# Autodesk Inventor assembly: T-Frame
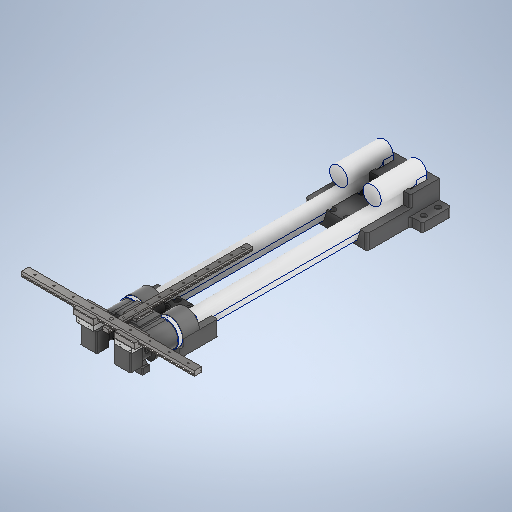
[picture p0: Inventor's stored thumbnail of the model, 512x512]
Saved by Autodesk Inventor 2026.2 (Build 302298010, 298A)
## iProperties
Created: 2026-03-27
Part Number: T-Frame
Document SubType Name: Assembly
Designer: chanh
Author: chanh
## Documents named in this file (15)
- C:\Users\chanh\내 드라이브\교과공부\2026년 1학기 (4학년 1학기)\01창의제품설계\CLOSE_hardware\02하체\도면\T-Frame.iam
- C:\Users\chanh\내 드라이브\교과공부\2026년 1학기 (4학년 1학기)\01창의제품설계\CLOSE_hardware\02하체\Linear Motor Bar (T-Frame).ipt
- C:\Users\chanh\내 드라이브\교과공부\2026년 1학기 (4학년 1학기)\01창의제품설계\CLOSE_hardware\02하체\Linear Motor (T-Frame).ipt
- C:\Users\chanh\내 드라이브\교과공부\2026년 1학기 (4학년 1학기)\01창의제품설계\CLOSE_hardware\02하체\Linear Motor Rear Braket.ipt
- C:\Users\chanh\내 드라이브\교과공부\2026년 1학기 (4학년 1학기)\01창의제품설계\CLOSE_hardware\02하체\Linear Motor Front Braket.ipt
- C:\Users\chanh\내 드라이브\교과공부\2026년 1학기 (4학년 1학기)\01창의제품설계\CLOSE_hardware\02하체\LMF20UU.ipt
- C:\Users\chanh\내 드라이브\교과공부\2026년 1학기 (4학년 1학기)\01창의제품설계\CLOSE_hardware\02하체\MGN15C Cart.ipt
- C:\Users\chanh\내 드라이브\교과공부\2026년 1학기 (4학년 1학기)\01창의제품설계\CLOSE_hardware\02하체\MGN15 Rail.ipt
- C:\Users\chanh\내 드라이브\교과공부\2026년 1학기 (4학년 1학기)\01창의제품설계\CLOSE_hardware\02하체\Linear Motor Mount Right.ipt
- C:\Users\chanh\내 드라이브\교과공부\2026년 1학기 (4학년 1학기)\01창의제품설계\CLOSE_hardware\02하체\Linear Motor Mount Left.ipt
- C:\Users\chanh\내 드라이브\교과공부\2026년 1학기 (4학년 1학기)\01창의제품설계\CLOSE_hardware\02하체\LM Cart Braket.ipt
- C:\Users\chanh\내 드라이브\교과공부\2026년 1학기 (4학년 1학기)\01창의제품설계\CLOSE_hardware\02하체\Space Craft Braket.ipt
- C:\Users\chanh\내 드라이브\교과공부\2026년 1학기 (4학년 1학기)\01창의제품설계\CLOSE_hardware\02하체\LM20UU.ipt
- C:\Users\chanh\내 드라이브\교과공부\2026년 1학기 (4학년 1학기)\01창의제품설계\CLOSE_hardware\02하체\MGN12C Cart.ipt
- C:\Users\chanh\내 드라이브\교과공부\2026년 1학기 (4학년 1학기)\01창의제품설계\CLOSE_hardware\02하체\MGN12 Rail.ipt
## Components (20 placed, 14 different names)
1. MGN15C Cart:1 — Slider:2, Rigid:8
2. MGN15 Rail:1 — Slider:1, Slider:2, Rotational:1
3. MGN15C Cart:2 — Slider:1, Flush:67, Flush:68, Mate:67
4. Linear Motor Mount Right:1 — Rigid:7, Mate:72
5. Linear Motor Mount Left:1 — Rigid:9, Mate:73
6. LM Cart Braket:1 — Flush:67, Flush:68, Mate:67, Mate:72
7. LM Cart Braket:2 — Rigid:8, Mate:73
8. Space Craft Braket:1 — Rigid:10, Rigid:11, Rigid:13
9. LM20UU:1 — Rigid:10, Mate:69
10. LM20UU:2 — Rigid:11, Mate:68
11. MGN12C Cart:1 — Rigid:13, Slider:3
12. MGN12 Rail:1 — Slider:3, Rotational:1
13. Linear Motor Front Braket:1 — Flush:56, Rigid:5, Rigid:6
14. LMF20UU:1 — Rigid:5
15. LMF20UU:2 — Rigid:6
16. Linear Motor (T-Frame):1 — Mate:32, Angle:2, T자 왼쪽 거리, Flush:53
17. Linear Motor Bar (T-Frame):1 — Mate:32, Angle:2, T자 왼쪽 거리, Rigid:7, Mate:69
18. Linear Motor (T-Frame):2 — T자 오른쪽 거리, Mate:34, Angle:3, Flush:54
19. Linear Motor Bar (T-Frame):2 — T자 오른쪽 거리, Mate:34, Angle:3, Rigid:9, Mate:68
20. Linear Motor Rear Braket:1 — Flush:53, Flush:54
## Relationships (29: Mate 9, WeldJoint 8, Flush 6, TranslationJoint 3, Angle 2, RevoluteJoint 1)
- T자 왼쪽 거리 [Mate] (84 mm): Linear Motor (T-Frame):1 ↔ Linear Motor Bar (T-Frame):1
- T자 오른쪽 거리 [Mate] (84 mm): Linear Motor (T-Frame):2 ↔ Linear Motor Bar (T-Frame):2
- Flush:1 (-240 mm)
- Mate:32: Linear Motor (T-Frame):1 ↔ Linear Motor Bar (T-Frame):1
- Angle:2 (-20 deg): Linear Motor (T-Frame):1 ↔ Linear Motor Bar (T-Frame):1
- Mate:34: Linear Motor (T-Frame):2 ↔ Linear Motor Bar (T-Frame):2
- Angle:3 (20 deg): Linear Motor (T-Frame):2 ↔ Linear Motor Bar (T-Frame):2
- Flush:53 (15 mm): Linear Motor (T-Frame):1 ↔ Linear Motor Rear Braket:1
- Flush:54 (15 mm): Linear Motor (T-Frame):2 ↔ Linear Motor Rear Braket:1
- Flush:56: Linear Motor Front Braket:1
- Rigid:5 [WeldJoint]: Linear Motor Front Braket:1 ↔ LMF20UU:1
- Rigid:6 [WeldJoint]: Linear Motor Front Braket:1 ↔ LMF20UU:2
- Slider:1 [TranslationJoint]: MGN15 Rail:1 ↔ MGN15C Cart:2
- Slider:2 [TranslationJoint]: MGN15C Cart:1 ↔ MGN15 Rail:1
- Rigid:7 [WeldJoint]: Linear Motor Mount Right:1 ↔ Linear Motor Bar (T-Frame):1
- Flush:67: MGN15C Cart:2 ↔ LM Cart Braket:1
- Flush:68: MGN15C Cart:2 ↔ LM Cart Braket:1
- Mate:67: MGN15C Cart:2 ↔ LM Cart Braket:1
- Rigid:8 [WeldJoint]: MGN15C Cart:1 ↔ LM Cart Braket:2
- Rigid:9 [WeldJoint]: Linear Motor Mount Left:1 ↔ Linear Motor Bar (T-Frame):2
- Rigid:10 [WeldJoint]: Space Craft Braket:1 ↔ LM20UU:1
- Rigid:11 [WeldJoint]: Space Craft Braket:1 ↔ LM20UU:2
- Mate:68: LM20UU:2 ↔ Linear Motor Bar (T-Frame):2
- Mate:69: LM20UU:1 ↔ Linear Motor Bar (T-Frame):1
- Rigid:13 [WeldJoint]: Space Craft Braket:1 ↔ MGN12C Cart:1
- Slider:3 [TranslationJoint]: MGN12C Cart:1 ↔ MGN12 Rail:1
- Rotational:1 [RevoluteJoint]: MGN15 Rail:1 ↔ MGN12 Rail:1
- Mate:72: Linear Motor Mount Right:1 ↔ LM Cart Braket:1
- Mate:73: Linear Motor Mount Left:1 ↔ LM Cart Braket:2
